# Autodesk Inventor assembly: AtwoodsAsmy
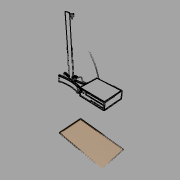
[picture p0: Inventor's stored thumbnail of the model, 180x180]
Saved by Autodesk Inventor 2012 SP2 (Build 160219200, 219)
## iProperties
Created: 2013-07-07
Part Number: AtwoodsAsmy
Document SubType Name: Assembly
Designer: 1
Author: 1
## Documents named in this file (9)
- D:\p3_metod1580library\figures\sources\M1-AtwoodsMachine\AtwoodsAsmy.iam
- D:\p3_metod1580library\figures\sources\M1-AtwoodsMachine\Atwoods-BaseBent.ipt
- D:\p3_metod1580library\figures\sources\M1-AtwoodsMachine\AdjLegStand.ipt
- D:\p3_metod1580library\figures\sources\M1-AtwoodsMachine\Ruler.ipt
- D:\p3_metod1580library\figures\sources\M1-AtwoodsMachine\BallHolder.ipt
- D:\p3_metod1580library\figures\sources\M1-AtwoodsMachine\BallReciever.ipt
- D:\p3_metod1580library\figures\sources\M1-AtwoodsMachine\AbstractBox.ipt
- D:\p3_metod1580library\figures\sources\M1-AtwoodsMachine\Atwoods-Wire1.ipt
- D:\p3_metod1580library\figures\sources\M1-AtwoodsMachine\Atwoods-Wire2.ipt
## Components (12 placed, 8 different names)
1. Atwoods-BaseBent:1 — Mate:1, Flush:1, Flush:2, Mate:2, Insert:3, Flush:3
2. Atwoods-BaseBent:2 — Mate:1, Flush:1, Flush:2, Insert:1, Insert:2
3. AdjLegStand:1 — Mate:2
4. AdjLegStand:2 — Insert:1
5. AdjLegStand:3 — Insert:2
6. AdjLegStand:4 — Insert:3
7. Ruler:1 — Flush:3, Flush:6, Flush:8
8. BallReciever:1 — Flush:6, Insert:4, Flush:8
9. BallHolder:1 — Insert:4
10. AbstractBox:1 — Flush:7, Flush:9, Flush:10, Flush:11, Flush:12
11. Atwoods-Wire1:1 — Flush:9, Flush:10, Flush:11
12. Atwoods-Wire2:1 — Flush:12
## Relationships (17: Flush 11, Insert 4, Mate 2)
- Mate:1: Atwoods-BaseBent:1 ↔ Atwoods-BaseBent:2
- Flush:1: Atwoods-BaseBent:1 ↔ Atwoods-BaseBent:2
- Flush:2: Atwoods-BaseBent:1 ↔ Atwoods-BaseBent:2
- Mate:2: Atwoods-BaseBent:1 ↔ AdjLegStand:1
- Insert:1: Atwoods-BaseBent:2 ↔ AdjLegStand:2
- Insert:2: Atwoods-BaseBent:2 ↔ AdjLegStand:3
- Insert:3: Atwoods-BaseBent:1 ↔ AdjLegStand:4
- Flush:3: Atwoods-BaseBent:1 ↔ Ruler:1
- Flush:6: Ruler:1 ↔ BallReciever:1
- Insert:4 (720 mm): BallReciever:1 ↔ BallHolder:1
- Flush:7: AbstractBox:1
- Flush:8: Ruler:1 ↔ BallReciever:1
- Flush:9: AbstractBox:1 ↔ Atwoods-Wire1:1
- Flush:10: AbstractBox:1 ↔ Atwoods-Wire1:1
- Flush:11: AbstractBox:1 ↔ Atwoods-Wire1:1
- Flush:12: AbstractBox:1 ↔ Atwoods-Wire2:1
- Flush:13 (-1000 mm)
